# Autodesk Inventor assembly: FifteenAssembly
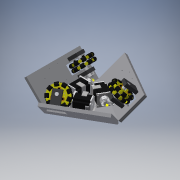
[picture p0: Inventor's stored thumbnail of the model, 180x180]
Saved by Autodesk Inventor 2016 (Build 200138000, 138)
## iProperties
Created: 2017-04-26
Part Number: FifteenAssembly
Document SubType Name: Assembly
Designer: Evan Phil George
Author: Evan Phil George
## Documents named in this file (9)
- C:\Users\Evan Phil George\Desktop\Ball Balancing Robot\TestBenchInventor\Acrylic Chassis\15mm\FifteenAssembly.iam
- C:\Users\Evan Phil George\Desktop\Ball Balancing Robot\TestBenchInventor\Acrylic Chassis\15mm\TraingleFifteen.ipt
- C:\Users\Evan Phil George\Desktop\Ball Balancing Robot\TestBenchInventor\Acrylic Chassis\15mm\RectangleFifteen1.ipt
- C:\Users\Evan Phil George\Desktop\Ball Balancing Robot\TestBenchInventor\Acrylic Chassis\15mm\RectangleFifteen2.ipt
- C:\Users\Evan Phil George\Desktop\Ball Balancing Robot\TestBenchInventor\Acrylic Chassis\15mm\RectangleFifteen3.ipt
- C:\Users\Evan Phil George\Desktop\Ball Balancing Robot\TestBenchInventor\SubAssemblies\MotorWithClamp.iam
- C:\Users\Evan Phil George\Desktop\Ball Balancing Robot\TestBenchInventor\SubAssemblies\MotorGear.iam
- C:\Users\Evan Phil George\Desktop\Ball Balancing Robot\TestBenchInventor\Acrylic Chassis\15mm\OmniSupport.ipt
- C:\Users\Evan Phil George\Desktop\Ball Balancing Robot\TestBenchInventor\SubAssemblies\OmniWheelGear.iam
## Components (19 placed, 19 different names)
1. TraingleFifteen:1 — Mate:1, Mate:2, Angle:1, Mate:3, Mate:4, Angle:2, Mate:5, Mate:6, Angle:3, Mate:7, Mate:8, Mate:9, Mate:26, Mate:27, Mate:28, Mate:33, Mate:34, Mate:35
2. RectangleFifteen1 — Mate:1, Mate:2, Angle:1, Mate:39, Mate:40, Mate:41, Mate:42, Mate:43, Mate:44
3. RectangleFifteen2 — Mate:3, Mate:4, Angle:2, Mate:20, Mate:21, Mate:22, Mate:23, Mate:24, Mate:25
4. RectangleFifteen3 — Mate:5, Mate:6, Angle:3, Mate:12, Mate:13, Mate:14, Mate:17, Mate:18, Mate:19
5. MotorWithClamp3 [sub-assembly] — Mate:7, Mate:8, Mate:9, Mate:10, Mate:11
6. MotorGear3 [sub-assembly] — Mate:10, Mate:11
7. OmniSupport3F — Mate:12, Mate:13, Mate:14, Mate:15, Mate:16
8. OmniWheelGear3 [sub-assembly] — Mate:15, Mate:16
9. OmniSupport3R — Mate:17, Mate:18, Mate:19
10. OmniSupport2F — Mate:20, Mate:21, Mate:22, Mate:31, Mate:32
11. OmniSupport2R — Mate:23, Mate:24, Mate:25
12. MotorWithClamp2 [sub-assembly] — Mate:26, Mate:27, Mate:28, Mate:29, Mate:38
13. MotorGear2 [sub-assembly] — Mate:29, Mate:38
14. OmniWheelGear:2 [sub-assembly] — Mate:31, Mate:32
15. MotorWithClamp1 [sub-assembly] — Mate:33, Mate:34, Mate:35, Mate:36, Mate:37
16. MotorGear1 [sub-assembly] — Mate:36, Mate:37
17. OmniWheelGear1 [sub-assembly] — Mate:45, Mate:46
18. OmniSupport1F — Mate:39, Mate:40, Mate:41, Mate:45, Mate:46
19. OmniSupport1R — Mate:42, Mate:43, Mate:44
## Relationships (48: Mate 45, Angle 3)
- Mate:1: TraingleFifteen:1 ↔ RectangleFifteen1
- Mate:2: TraingleFifteen:1 ↔ RectangleFifteen1
- Angle:1 (45 deg): TraingleFifteen:1 ↔ RectangleFifteen1
- Mate:3: TraingleFifteen:1 ↔ RectangleFifteen2
- Mate:4: TraingleFifteen:1 ↔ RectangleFifteen2
- Angle:2 (45 deg): TraingleFifteen:1 ↔ RectangleFifteen2
- Mate:5: TraingleFifteen:1 ↔ RectangleFifteen3
- Mate:6: TraingleFifteen:1 ↔ RectangleFifteen3
- Angle:3 (45 deg): TraingleFifteen:1 ↔ RectangleFifteen3
- Mate:7: TraingleFifteen:1 ↔ MotorWithClamp3
- Mate:8: TraingleFifteen:1 ↔ MotorWithClamp3
- Mate:9: TraingleFifteen:1 ↔ MotorWithClamp3
- Mate:10: MotorWithClamp3 ↔ MotorGear3
- Mate:11: MotorWithClamp3 ↔ MotorGear3
- Mate:12: RectangleFifteen3 ↔ OmniSupport3F
- Mate:13: RectangleFifteen3 ↔ OmniSupport3F
- Mate:14: RectangleFifteen3 ↔ OmniSupport3F
- Mate:15: OmniSupport3F ↔ OmniWheelGear3
- Mate:16 (0.25 mm): OmniSupport3F ↔ OmniWheelGear3
- Mate:17: RectangleFifteen3 ↔ OmniSupport3R
- Mate:18: RectangleFifteen3 ↔ OmniSupport3R
- Mate:19: RectangleFifteen3 ↔ OmniSupport3R
- Mate:20: RectangleFifteen2 ↔ OmniSupport2F
- Mate:21: RectangleFifteen2 ↔ OmniSupport2F
- Mate:22: RectangleFifteen2 ↔ OmniSupport2F
- Mate:23: RectangleFifteen2 ↔ OmniSupport2R
- Mate:24: RectangleFifteen2 ↔ OmniSupport2R
- Mate:25: RectangleFifteen2 ↔ OmniSupport2R
- Mate:26: TraingleFifteen:1 ↔ MotorWithClamp2
- Mate:27: TraingleFifteen:1 ↔ MotorWithClamp2
- Mate:28: TraingleFifteen:1 ↔ MotorWithClamp2
- Mate:29: MotorWithClamp2 ↔ MotorGear2
- Mate:31: OmniSupport2F ↔ OmniWheelGear:2
- Mate:32 (0.25 mm): OmniSupport2F ↔ OmniWheelGear:2
- Mate:33: TraingleFifteen:1 ↔ MotorWithClamp1
- Mate:34: TraingleFifteen:1 ↔ MotorWithClamp1
- Mate:35: TraingleFifteen:1 ↔ MotorWithClamp1
- Mate:36: MotorWithClamp1 ↔ MotorGear1
- Mate:37: MotorWithClamp1 ↔ MotorGear1
- Mate:38: MotorWithClamp2 ↔ MotorGear2
- Mate:39: RectangleFifteen1 ↔ OmniSupport1F
- Mate:40: RectangleFifteen1 ↔ OmniSupport1F
- Mate:41: RectangleFifteen1 ↔ OmniSupport1F
- Mate:42: RectangleFifteen1 ↔ OmniSupport1R
- Mate:43: RectangleFifteen1 ↔ OmniSupport1R
- Mate:44: RectangleFifteen1 ↔ OmniSupport1R
- Mate:45: OmniWheelGear1 ↔ OmniSupport1F
- Mate:46 (0.25 mm): OmniWheelGear1 ↔ OmniSupport1F
